# Autodesk Inventor assembly: Weapon Stack
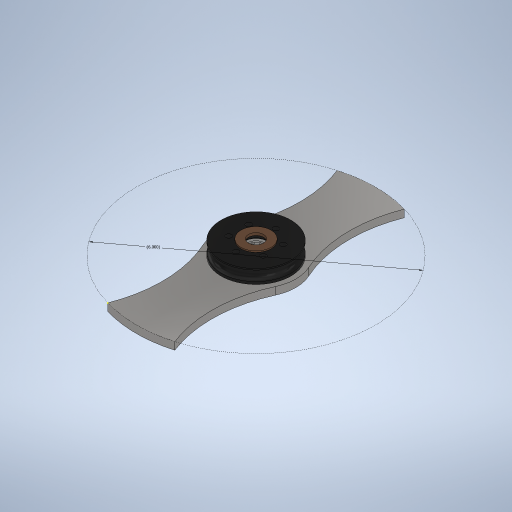
[picture p0: Inventor's stored thumbnail of the model, 512x512]
Saved by Autodesk Inventor 2023.2 (Build 272271000, 271)
## iProperties
Created: 2022-11-18
Part Number: Weapon Stack
Document SubType Name: Assembly
Designer: Nathan Cai
Mass: 219.513 g
Surface Area: 160.182 cm^2
Volume: 27.3653 cm^3
Density: 8.0216 g/cm^3
Author: Nathan Cai
## Documents named in this file (6)
- E:\Documents\Inventor\0.3rd Lawette - V3.5\Horizontal Weapon Assembly (Type FD)\Weapon Stack.iam
- E:\Documents\Inventor\0.3rd Lawette - V3.5\Horizontal Weapon Assembly (Type FD)\Blade (Bar 2).ipt
- E:\Documents\Inventor\0.3rd Lawette - V3.5\Horizontal Weapon Assembly (Type FD)\7421K2_Ultra-Low-Friction Oil-Embedded Thrust Bearing.ipt
- E:\Documents\Inventor\0.3rd Lawette - V3.5\Horizontal Weapon Assembly (Type FD)\5905K497_Needle-Roller Bearing.ipt
- E:\Documents\Inventor\0.3rd Lawette - V3.5\Horizontal Weapon Assembly (Type FD)\Weapon Pulley.ipt
- E:\Documents\Inventor\0.3rd Lawette - V3.5\Horizontal Weapon Assembly (Type FD)\Weapon Cover.ipt
## Components (6 placed, 5 different names)
1. Blade (Bar 2):1 — Mate:1, Mate:2, Mate:4, Mate:8, Mate:9, Mate:11, Mate:12
2. 7421K2_Ultra-Low-Friction Oil-Embedded Thrust Bearing:1 — Mate:1, Mate:2, Mate:3, Mate:10
3. 5905K497_Needle-Roller Bearing:1 — Mate:3, Mate:4, Mate:5, Mate:6, Mate:7
4. 7421K2_Ultra-Low-Friction Oil-Embedded Thrust Bearing:2 — Mate:5, Mate:6
5. Weapon Pulley:1 — Mate:7, Mate:8, Mate:9
6. Weapon Cover:1 — Mate:10, Mate:11, Mate:12
## Relationships (12: Mate 12)
- Mate:1: Blade (Bar 2):1 ↔ 7421K2_Ultra-Low-Friction Oil-Embedded Thrust Bearing:1
- Mate:2: Blade (Bar 2):1 ↔ 7421K2_Ultra-Low-Friction Oil-Embedded Thrust Bearing:1
- Mate:3: 7421K2_Ultra-Low-Friction Oil-Embedded Thrust Bearing:1 ↔ 5905K497_Needle-Roller Bearing:1
- Mate:4: Blade (Bar 2):1 ↔ 5905K497_Needle-Roller Bearing:1
- Mate:5 (3.175 mm): 5905K497_Needle-Roller Bearing:1 ↔ 7421K2_Ultra-Low-Friction Oil-Embedded Thrust Bearing:2
- Mate:6: 5905K497_Needle-Roller Bearing:1 ↔ 7421K2_Ultra-Low-Friction Oil-Embedded Thrust Bearing:2
- Mate:7: 5905K497_Needle-Roller Bearing:1 ↔ Weapon Pulley:1
- Mate:8: Blade (Bar 2):1 ↔ Weapon Pulley:1
- Mate:9: Blade (Bar 2):1 ↔ Weapon Pulley:1
- Mate:10: 7421K2_Ultra-Low-Friction Oil-Embedded Thrust Bearing:1 ↔ Weapon Cover:1
- Mate:11: Blade (Bar 2):1 ↔ Weapon Cover:1
- Mate:12: Blade (Bar 2):1 ↔ Weapon Cover:1
